# Autodesk Inventor assembly: Dynamixel MX-64T
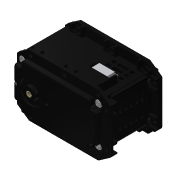
[picture p0: Inventor's stored thumbnail of the model, 180x180]
Saved by Autodesk Inventor 2019 (Build 230136000, 136)
## iProperties
Created: 2021-10-16
Part Number: Dynamixel MX-64T
Document SubType Name: Assembly
Designer: user
Author: user
## Documents named in this file (5)
- E:\Robotika\KRPAI\Project 2021\Dynamixel MX-64\Dynamixel MX-64T.iam
- E:\Robotika\KRPAI\Project 2021\Dynamixel MX-64\Belakang.ipt
- E:\Robotika\KRPAI\Project 2021\Dynamixel MX-64\Depan.ipt
- E:\Robotika\KRPAI\Project 2021\Dynamixel MX-64\Tengah.ipt
- E:\Robotika\KRPAI\Project 2021\Dynamixel MX-64\Kepala Baut.ipt
## Components (7 placed, 4 different names)
1. Belakang:1 — Mate:1, Mate:3, Flush:1, Mate:5, Mate:6, Mate:7, Mate:8, Mate:9, Mate:10, Mate:11, Mate:12
2. Depan:1 — Mate:2, Mate:4, Flush:2
3. Tengah:1 — Mate:1, Mate:2, Mate:3, Mate:4, Flush:1, Flush:2
4. Kepala Baut:1 — Mate:9, Mate:12
5. Kepala Baut:2 — Mate:7, Mate:10
6. Kepala Baut:3 — Mate:5, Mate:6
7. Kepala Baut:4 — Mate:8, Mate:11
## Relationships (14: Mate 12, Flush 2)
- Mate:1: Belakang:1 ↔ Tengah:1
- Mate:2: Depan:1 ↔ Tengah:1
- Mate:3: Belakang:1 ↔ Tengah:1
- Mate:4: Depan:1 ↔ Tengah:1
- Flush:1: Belakang:1 ↔ Tengah:1
- Flush:2: Depan:1 ↔ Tengah:1
- Mate:5: Belakang:1 ↔ Kepala Baut:3
- Mate:6: Belakang:1 ↔ Kepala Baut:3
- Mate:7: Belakang:1 ↔ Kepala Baut:2
- Mate:8: Belakang:1 ↔ Kepala Baut:4
- Mate:9: Belakang:1 ↔ Kepala Baut:1
- Mate:10: Belakang:1 ↔ Kepala Baut:2
- Mate:11: Belakang:1 ↔ Kepala Baut:4
- Mate:12: Belakang:1 ↔ Kepala Baut:1
